# Autodesk Inventor assembly: Assembly
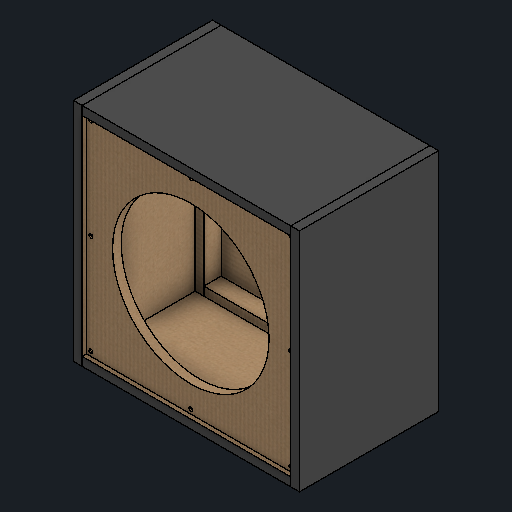
[picture p0: Inventor's stored thumbnail of the model, 512x512]
Saved by Autodesk Inventor 2026.2 (Build 302298000, 298)
## iProperties
Created: 2026-06-16
Part Number: Assembly
Document SubType Name: Assembly
Designer: JoshuaEah
Author: JoshuaEah
## Documents named in this file (6)
- C:\Users\JoshuaEah\Documents\GitHub\Designed-Trinkets\Guitar\110 Guitar Cab\Assembly.iam
- C:\Users\JoshuaEah\Documents\GitHub\Designed-Trinkets\Guitar\110 Guitar Cab\Back Plate.ipt
- C:\Users\JoshuaEah\Documents\GitHub\Designed-Trinkets\Guitar\110 Guitar Cab\Bracing.iam
- C:\Users\JoshuaEah\Documents\GitHub\Designed-Trinkets\Guitar\110 Guitar Cab\Front Baffle.ipt
- C:\Users\JoshuaEah\Documents\GitHub\Designed-Trinkets\Guitar\110 Guitar Cab\Side Panel.ipt
- C:\Users\JoshuaEah\Documents\GitHub\Designed-Trinkets\Guitar\110 Guitar Cab\Top and Bottom Panel.ipt
## Components (9 placed, 5 different names)
1. Top and Bottom Panel:1 — Mate:1, Flush:1, Flush:2, Mate:2, Flush:3, Flush:4, Flush:10, Mate:16, Flush:15
2. Top and Bottom Panel:2 — Flush:5, Flush:6, Mate:3
3. Side Panel:1 — Mate:1, Flush:1, Flush:2, Flush:5, Flush:6, Mate:3, Mate:17
4. Side Panel:2 — Mate:2, Flush:3, Flush:4
5. Front Baffle — Mate:20, Flush:16, Flush:17
6. Bracing:1 [sub-assembly] — Flush:15, Mate:20, Flush:16, Flush:17
7. Bracing:2 [sub-assembly] — Flush:10, Mate:16, Mate:17, Mate:18, Flush:11, Flush:12, Mate:19, Flush:13, Flush:14
8. Back Plate:1 — Mate:18, Flush:11, Flush:12
9. Back Plate:2 — Mate:19, Flush:13, Flush:14
## Relationships (26: Flush 14, Mate 12)
- Mate:1: Top and Bottom Panel:1 ↔ Side Panel:1
- Flush:1: Top and Bottom Panel:1 ↔ Side Panel:1
- Flush:2: Top and Bottom Panel:1 ↔ Side Panel:1
- Mate:2: Top and Bottom Panel:1 ↔ Side Panel:2
- Flush:3: Top and Bottom Panel:1 ↔ Side Panel:2
- Flush:4: Top and Bottom Panel:1 ↔ Side Panel:2
- Flush:5: Top and Bottom Panel:2 ↔ Side Panel:1
- Flush:6: Top and Bottom Panel:2 ↔ Side Panel:1
- Mate:3: Top and Bottom Panel:2 ↔ Side Panel:1
- [Mate]: Side Panel:1 ↔ Bracing:1
- [Mate]: Top and Bottom Panel:1 ↔ Bracing:1
- [Mate]: Top and Bottom Panel:1 ↔ Bracing:1
- [Mate]: Side Panel:2 ↔ Bracing:1
- Flush:10 (12.7 mm): Top and Bottom Panel:1 ↔ Bracing:2
- Mate:16: Top and Bottom Panel:1 ↔ Bracing:2
- Mate:17: Side Panel:1 ↔ Bracing:2
- Mate:18: Bracing:2 ↔ Back Plate:1
- Flush:11: Bracing:2 ↔ Back Plate:1
- Flush:12: Bracing:2 ↔ Back Plate:1
- Mate:19: Bracing:2 ↔ Back Plate:2
- Flush:13: Bracing:2 ↔ Back Plate:2
- Flush:14: Bracing:2 ↔ Back Plate:2
- Flush:15 (19.05 mm): Top and Bottom Panel:1 ↔ Bracing:1
- Mate:20: Front Baffle ↔ Bracing:1
- Flush:16: Front Baffle ↔ Bracing:1
- Flush:17: Front Baffle ↔ Bracing:1
## Named parameters: Finish1_Area = 3468.91, Finish1_Thickness = 0.05 mm
note: some values were not read from the file. Shown as the stored number, unit unknown: "Finish1_Area".
